# Autodesk Inventor assembly: 总1
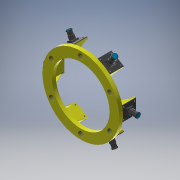
[picture p0: Inventor's stored thumbnail of the model, 180x180]
Saved by Autodesk Inventor 2017 (Build 210142000, 142)
## iProperties
Part Number: 总1
Material: 常规
Document SubType Name: Assembly
Designer: Administrator
Author: Administrator
## Documents named in this file (6)
- D:\大四上\传感器\小轿车\总1.iam
- D:\大四上\传感器\小轿车\镜头.ipt
- D:\大四上\传感器\小轿车\相机.ipt
- D:\大四上\传感器\小轿车\支座.ipt
- C:\Users\Administrator\Documents\Inventor\Content Center Files\R2017\zh-CN\GB_T 70.1\螺钉 GB_T 70.1 M1.6 x 8.ipt
- C:\Users\Administrator\Documents\Inventor\Content Center Files\R2017\zh-CN\GB_T 6170-2000\螺母 GB_T 6170 M1.6.ipt
## Components (61 placed, 5 different names)
1. 支座:1 — 配合:7, 配合:8, 配合:9, 配合:10, 配合:11, 配合:12, 配合:13, 配合:14, 配合:15, 插入:5, 插入:6, 插入:7, 插入:8
2. 相机:3 — 配合:7, 配合:8, 配合:9
3. 镜头:3
4. 相机:2 — 配合:10, 配合:11, 配合:12, 插入:1, 插入:2, 插入:3, 插入:4
5. 镜头:2
6. 相机:1 — 配合:1, 配合:2, 配合:13, 配合:14, 配合:15
7. 镜头:1 — 配合:1, 配合:2
8. 相机:4
9. 镜头:4
10. 相机:5
11. 镜头:5
12. 相机:6
13. 镜头:6
14. 螺钉 GB/T 70.1 M1.6 x 8:1 — 插入:1
15. 螺钉 GB/T 70.1 M1.6 x 8:2 — 插入:2
16. 螺钉 GB/T 70.1 M1.6 x 8:3 — 插入:3
17. 螺钉 GB/T 70.1 M1.6 x 8:4 — 插入:4
18. 螺母 GB/T 6170-2000 M1.6:1 — 插入:5
19. 螺母 GB/T 6170-2000 M1.6:2 — 插入:6
20. 螺母 GB/T 6170-2000 M1.6:3 — 插入:7
21. 螺母 GB/T 6170-2000 M1.6:4 — 插入:8
22. 螺钉 GB/T 70.1 M1.6 x 8:5
23. 螺钉 GB/T 70.1 M1.6 x 8:6
24. 螺钉 GB/T 70.1 M1.6 x 8:7
25. 螺钉 GB/T 70.1 M1.6 x 8:8
26. 螺母 GB/T 6170-2000 M1.6:5
27. 螺母 GB/T 6170-2000 M1.6:6
28. 螺母 GB/T 6170-2000 M1.6:7
29. 螺母 GB/T 6170-2000 M1.6:8
30. 螺钉 GB/T 70.1 M1.6 x 8:9
31. 螺钉 GB/T 70.1 M1.6 x 8:10
32. 螺钉 GB/T 70.1 M1.6 x 8:11
33. 螺钉 GB/T 70.1 M1.6 x 8:12
34. 螺母 GB/T 6170-2000 M1.6:9
35. 螺母 GB/T 6170-2000 M1.6:10
36. 螺母 GB/T 6170-2000 M1.6:11
37. 螺母 GB/T 6170-2000 M1.6:12
38. 螺钉 GB/T 70.1 M1.6 x 8:13
39. 螺钉 GB/T 70.1 M1.6 x 8:14
40. 螺钉 GB/T 70.1 M1.6 x 8:15
41. 螺钉 GB/T 70.1 M1.6 x 8:16
42. 螺母 GB/T 6170-2000 M1.6:13
43. 螺母 GB/T 6170-2000 M1.6:14
44. 螺母 GB/T 6170-2000 M1.6:15
45. 螺母 GB/T 6170-2000 M1.6:16
46. 螺钉 GB/T 70.1 M1.6 x 8:17
47. 螺钉 GB/T 70.1 M1.6 x 8:18
48. 螺钉 GB/T 70.1 M1.6 x 8:19
49. 螺钉 GB/T 70.1 M1.6 x 8:20
50. 螺母 GB/T 6170-2000 M1.6:17
51. 螺母 GB/T 6170-2000 M1.6:18
52. 螺母 GB/T 6170-2000 M1.6:19
53. 螺母 GB/T 6170-2000 M1.6:20
54. 螺钉 GB/T 70.1 M1.6 x 8:21
55. 螺钉 GB/T 70.1 M1.6 x 8:22
56. 螺钉 GB/T 70.1 M1.6 x 8:23
57. 螺钉 GB/T 70.1 M1.6 x 8:24
58. 螺母 GB/T 6170-2000 M1.6:21
59. 螺母 GB/T 6170-2000 M1.6:22
60. 螺母 GB/T 6170-2000 M1.6:23
61. 螺母 GB/T 6170-2000 M1.6:24
## Component patterns: (2 elements, first: 相机:3 + 镜头:3 + 相机:2 + 镜头:2 + 相机:1 + 镜头:1), (3 elements, first: 螺钉 GB/T 70.1 M1.6 x 8:1 + 螺钉 GB/T 70.1 M1.6 x 8:2 + 螺钉 GB/T 70.1 M1.6 x 8:3 + 螺钉 GB/T 70.1 M1.6 x 8:4 + 螺母 GB/T 6170-2000 M1.6:1 + 螺母 GB/T 6170-2000 M1.6:2 + 螺母 GB/T 6170-2000 M1.6:3 + 螺母 GB/T 6170-2000 M1.6:4), 零部件阵列 1:2 (3 elements)
## Relationships (23: Mate 15, Insert 8)
- 配合:1 [Mate]: 相机:1 ↔ 镜头:1
- 配合:2 [Mate]: 相机:1 ↔ 镜头:1
- [Mate]: 相机:2 ↔ 镜头:2
- [Mate]: 相机:2 ↔ 镜头:2
- [Mate]: 相机:3 ↔ 镜头:3
- [Mate]: 相机:3 ↔ 镜头:3
- 配合:7 [Mate]: 支座:1 ↔ 相机:3
- 配合:8 [Mate]: 支座:1 ↔ 相机:3
- 配合:9 [Mate]: 支座:1 ↔ 相机:3
- 配合:10 [Mate]: 支座:1 ↔ 相机:2
- 配合:11 [Mate]: 支座:1 ↔ 相机:2
- 配合:12 [Mate]: 支座:1 ↔ 相机:2
- 配合:13 [Mate]: 支座:1 ↔ 相机:1
- 配合:14 [Mate]: 支座:1 ↔ 相机:1
- 配合:15 [Mate]: 支座:1 ↔ 相机:1
- 插入:1 [Insert]: 相机:2 ↔ 螺钉 GB/T 70.1 M1.6 x 8:1
- 插入:2 [Insert]: 相机:2 ↔ 螺钉 GB/T 70.1 M1.6 x 8:2
- 插入:3 [Insert]: 相机:2 ↔ 螺钉 GB/T 70.1 M1.6 x 8:3
- 插入:4 [Insert]: 相机:2 ↔ 螺钉 GB/T 70.1 M1.6 x 8:4
- 插入:5 [Insert]: 支座:1 ↔ 螺母 GB/T 6170-2000 M1.6:1
- 插入:6 [Insert]: 支座:1 ↔ 螺母 GB/T 6170-2000 M1.6:2
- 插入:7 [Insert]: 支座:1 ↔ 螺母 GB/T 6170-2000 M1.6:3
- 插入:8 [Insert]: 支座:1 ↔ 螺母 GB/T 6170-2000 M1.6:4
## Named parameters: d2_d0 = 0 mm, d3_d1 = 0 mm, d4_d0 = 0 mm, d5_d1 = 0 mm
